# Autodesk Inventor assembly: 1376.000(1)
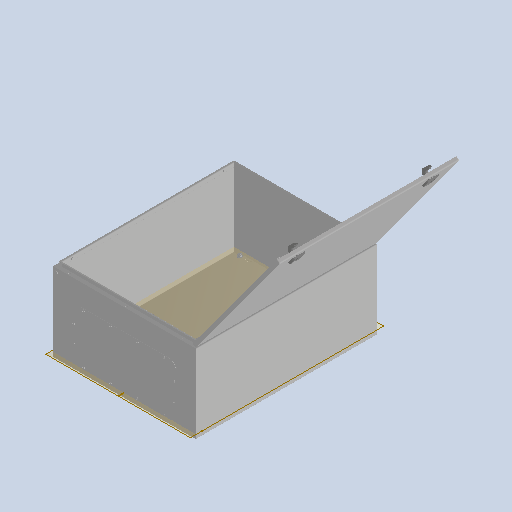
[picture p0: Inventor's stored thumbnail of the model, 512x512]
Saved by Autodesk Inventor 2025.2 (Build 292293000, 293)
## iProperties
Created: 2025-05-05
Part Number: 1376.000(1)
Catalog Web Link: www.cadenas.de
Description: AX Compact enclosure-sheet steel
Vendor: RITTAL
Document SubType Name: Assembly
Designer: psAdmin
Manufacturer: RITTAL
Mass: 34000 g
Surface Area: 49007 cm^2
Volume: 4441.12 cm^3
Density: 7.65572 g/cm^3
Category: PARTsolutions
Company: RITTAL
PSOL_IDENT_0: {$CADENAS_DATA/23d-libs/rittal/schaltschranksys/kompakt_schaltschr/ae_2_0_asmtab.prj},203 {VTYP=3D},
PSOL_IDENT_1: {STYP=ASSTAB},{NB=1376.000(1)},{LINA=1376.000(1)},{NN=AX Compact enclosure},{DATE=28.04.2025 21:11:2
PSOL_IDENT_2: 3},{GEOMDATE=11.04.2025 11:21:44},{VERSION=},{LINEID=320},{WBVAR=DETAIL},{WBNUMERIC=DETAIL}  {NB=137
PSOL_IDENT_3: 6.000(1)},{LINA=1376.000(1)},{KT=DUMMY},{BEST=1376.000},{BEM=2},{DETAIL=1},{INFOWWW=Website},{BEZ1=A
PSOL_IDENT_4: X Kompakt-Schaltschrank},{BEZ2=Stahlblech},{BEZ3=eintürig},{INFO=Überarbeitete Version 11/2024},{B=6
PSOL_IDENT_5: 00},{H=760},{T=350},{F=550},{G=735},{B1=600},{H1=760},{T1=350},{F1=550},{G1=735},{S=3.0},{ST=MIN},{G
PSOL_IDENT_6: EW=34},{VERS=19},{CNSECLASS51=27-18-01-02},{CNSECLASS70=27-18-01-01},{CNSECLASS80=27-18-01-01},{CNSE
PSOL_IDENT_7: TIM40=EC000261},{PPATH=assemblies_ae_2_0/ae_2_0_asmtpl.prj},{INFOPAGE=ax_s30},{INFOPATH=http://www.r
PSOL_IDENT_8: ittal.com/de-de/part/1376000},{BESTE1=1376},{BESTE2=000},{DETAIL1= 2, 'niedrig', 'detail_2.png', 1, '
PSOL_IDENT_9: hoch', 'detail_1.png', 11  , 'hochsperr', 'detail_11.png'},{CNSETIM80=EC000261},{CNSETIM90=EC000261}
PSOL_IDENT_10: ,{CNSECLASS60=27-18-01-01},{UNSPSC=31-26-15-02}
NB: 1376.000(1)
NN: AX Compact enclosure
NT: sheet steel
NBSYN: $BEST.($DETAIL.)
LINA: 1376.000(1)
CATALOG: Rittal
BEST: 1376.000
DETAIL: high
INFOWWW: webseite
BEZ1: AX Compact enclosure
BEZ2: sheet steel
BEZ3: single door
INFO: Revised version 11/2024
B: 600
H: 760
T: 350
F: 550
G: 735
GEW: 34
CNSECLASS70: 27-18-01-01
CNSECLASS80: 27-18-01-01
CNSETIM80: EC000261
CNSETIM90: EC000261
CNSECLASS60: 27-18-01-01
UNSPSC: 31-26-15-02
SUPPLIER: RITTAL
ARTICLENO: 1376.000(1)
BOMINFO: 1376.000(1)
CREATOR: CADENAS GmbH
Title: 1376.000(1)
Author: Cadenas PARTsolutions
Comments: sheet steel
## Documents named in this file (13)
- C:\Users\lucas\OneDrive\Documentos\Documentos\Gustavo\Mozangao\Projeto Base (5140)\Q.E - Braço Robotico\Q.E Rital\AIS2024\1376_000_1_\1376_000(1).iam
- C:\Users\lucas\OneDrive\Documentos\Documentos\Gustavo\Mozangao\Projeto Base (5140)\Q.E - Braço Robotico\Q.E Rital\AIS2024\1376_000_1_\1376_000(1)_P1.ipt
- C:\Users\lucas\OneDrive\Documentos\Documentos\Gustavo\Mozangao\Projeto Base (5140)\Q.E - Braço Robotico\Q.E Rital\AIS2024\1376_000_1_\1XXX_01_04(B,1)_P7.ipt
- C:\Users\lucas\OneDrive\Documentos\Documentos\Gustavo\Mozangao\Projeto Base (5140)\Q.E - Braço Robotico\Q.E Rital\AIS2024\1376_000_1_\1XXX_01_04(T,1)_P7.ipt
- C:\Users\lucas\OneDrive\Documentos\Documentos\Gustavo\Mozangao\Projeto Base (5140)\Q.E - Braço Robotico\Q.E Rital\AIS2024\1376_000_1_\1676X_01_01(1)_P2.ipt
- C:\Users\lucas\OneDrive\Documentos\Documentos\Gustavo\Mozangao\Projeto Base (5140)\Q.E - Braço Robotico\Q.E Rital\AIS2024\1376_000_1_\6321_050_P9 1.ipt
- C:\Users\lucas\OneDrive\Documentos\Documentos\Gustavo\Mozangao\Projeto Base (5140)\Q.E - Braço Robotico\Q.E Rital\AIS2024\1376_000_1_\1XXX_01_05(1)_P8.ipt
- C:\Users\lucas\OneDrive\Documentos\Documentos\Gustavo\Mozangao\Projeto Base (5140)\Q.E - Braço Robotico\Q.E Rital\AIS2024\1376_000_1_\0000-00186369(1).ipt
- C:\Users\lucas\OneDrive\Documentos\Documentos\Gustavo\Mozangao\Projeto Base (5140)\Q.E - Braço Robotico\Q.E Rital\AIS2024\1376_000_1_\1XX1_04_00_1(1)_P5.ipt
- C:\Users\lucas\OneDrive\Documentos\Documentos\Gustavo\Mozangao\Projeto Base (5140)\Q.E - Braço Robotico\Q.E Rital\AIS2024\1376_000_1_\0000-00082819_P2.ipt
- C:\Users\lucas\OneDrive\Documentos\Documentos\Gustavo\Mozangao\Projeto Base (5140)\Q.E - Braço Robotico\Q.E Rital\AIS2024\1376_000_1_\1676X_02_00_P6_(1).ipt
- C:\Users\lucas\OneDrive\Documentos\Documentos\Gustavo\Mozangao\Projeto Base (5140)\Q.E - Braço Robotico\Q.E Rital\AIS2024\1376_000_1_\0000-00168553(1).ipt
- C:\Users\lucas\OneDrive\Documentos\Documentos\Gustavo\Mozangao\Projeto Base (5140)\Q.E - Braço Robotico\Q.E Rital\AIS2024\1376_000_1_\0000-00189079(1).ipt
## Components (28 placed, 12 different names)
1. 1376_000(1)_P1:1 — SCRO_XY@1 <-> SC_XY@2, SCRO_Z@1 <-> SC_Z@2, SCRO_YZ@1 <-> SC_YZ@2, SCRU_XY@1 <-> SC_XY@3, SCRU_Z@1 <-> SC_Z@3, SCRU_YZ@1 <-> SC_YZ@3, SCLO_XY@1 <-> Hinge_Plug_XY@8, SCLO_Z@1 <-> Hinge_Plug_Z@8, SCLO_YZ@1 <-> Hinge_Plug_YZ@8, SCLU_XY@1 <-> Hinge_Plug_XY@9, SCLU_Z@1 <-> Hinge_Plug_Z@9, SCLU_YZ@1 <-> Hinge_Plug_YZ@9, FP1_XY@1 <-> FP_XY@10, FP1_Z@1 <-> FP_Z@10, FP1_YZ@1 <-> FP_YZ@10, MP_XY@1 <-> MP_XY@23, MP_Z@1 <-> MP_Z@23, MP_YZ@1 <-> MP_YZ@23, to_Plug_XY@1 <-> P1_XY@24, to_Plug_Z@1 <-> P1_Z@24, to_Plug_YZ@1 <-> P1_YZ@24, to_Cap_1_XY@1 <-> CAP_XY@25, to_Cap_1_Z@1 <-> CAP_Z@25, to_Cap_1_YZ@1 <-> CAP_YZ@25, to_Cap_2_XY@1 <-> CAP_XY@26, to_Cap_2_Z@1 <-> CAP_Z@26, to_Cap_2_YZ@1 <-> CAP_YZ@26, to_Cap_3_XY@1 <-> CAP_XY@27, to_Cap_3_Z@1 <-> CAP_Z@27, to_Cap_3_YZ@1 <-> CAP_YZ@27, to_Cap_4_XY@1 <-> CAP_XY@28, to_Cap_4_Z@1 <-> CAP_Z@28, to_Cap_4_YZ@1 <-> CAP_YZ@28
2. 1XXX_01_04(B,1)_P7:1 — SCRO_XY@1 <-> SC_XY@2, SCRO_Z@1 <-> SC_Z@2, SCRO_YZ@1 <-> SC_YZ@2
3. 1XXX_01_04(T,1)_P7:1 — SCRU_XY@1 <-> SC_XY@3, SCRU_Z@1 <-> SC_Z@3, SCRU_YZ@1 <-> SC_YZ@3, TUER2_XY@3 <-> ET_XY@4, TUER2_Z@3 <-> ET_Z@4
4. 1676X_01_01(1)_P2:1 — TUER2_XY@3 <-> ET_XY@4, TUER2_Z@3 <-> ET_Z@4, to_Auflaufelement_XY@4 <-> P9_XY@5, to_Auflaufelement_Z@4 <-> P9_Z@5, to_Auflaufelement_YZ@4 <-> P9_YZ@5, VV1_XY@4 <-> VV_XY@6, VV1_Z@4 <-> VV_Z@6, VV1_YZ@4 <-> VV_YZ@6, VV2_XY@4 <-> VV_XY@7, VV2_Z@4 <-> VV_Z@7, VV2_YZ@4 <-> VV_YZ@7
5. 6321_050_P9 1:1 — to_Auflaufelement_XY@4 <-> P9_XY@5, to_Auflaufelement_Z@4 <-> P9_Z@5, to_Auflaufelement_YZ@4 <-> P9_YZ@5
6. 1XXX_01_05(1)_P8:1 — VV1_XY@4 <-> VV_XY@6, VV1_Z@4 <-> VV_Z@6, VV1_YZ@4 <-> VV_YZ@6
7. 1XXX_01_05(1)_P8:2 — VV2_XY@4 <-> VV_XY@7, VV2_Z@4 <-> VV_Z@7, VV2_YZ@4 <-> VV_YZ@7
8. 0000-00186369(1):1 — SCLO_XY@1 <-> Hinge_Plug_XY@8, SCLO_Z@1 <-> Hinge_Plug_Z@8, SCLO_YZ@1 <-> Hinge_Plug_YZ@8
9. 0000-00186369(1):2 — SCLU_XY@1 <-> Hinge_Plug_XY@9, SCLU_Z@1 <-> Hinge_Plug_Z@9, SCLU_YZ@1 <-> Hinge_Plug_YZ@9
10. 1XX1_04_00_1(1)_P5:1 — FP1_XY@1 <-> FP_XY@10, FP1_Z@1 <-> FP_Z@10, FP1_YZ@1 <-> FP_YZ@10, to_Bolt_1_XY@10 <-> Bolt_XY@11, to_Bolt_1_Z@10 <-> Bolt_Z@11, to_Bolt_1_YZ@10 <-> Bolt_YZ@11, to_Bolt_2_XY@10 <-> Bolt_XY@12, to_Bolt_2_Z@10 <-> Bolt_Z@12, to_Bolt_2_YZ@10 <-> Bolt_YZ@12, to_Bolt_3_XY@10 <-> Bolt_XY@13, to_Bolt_3_Z@10 <-> Bolt_Z@13, to_Bolt_3_YZ@10 <-> Bolt_YZ@13, to_Bolt_4_XY@10 <-> Bolt_XY@14, to_Bolt_4_Z@10 <-> Bolt_Z@14, to_Bolt_4_YZ@10 <-> Bolt_YZ@14, to_Bolt_1_1_XY@10 <-> Bolt_XY@15, to_Bolt_1_1_Z@10 <-> Bolt_Z@15, to_Bolt_1_1_YZ@10 <-> Bolt_YZ@15, to_Bolt_1_2_XY@10 <-> Bolt_XY@16, to_Bolt_1_2_Z@10 <-> Bolt_Z@16, to_Bolt_1_2_YZ@10 <-> Bolt_YZ@16, to_Bolt_1_3_XY@10 <-> Bolt_XY@17, to_Bolt_1_3_Z@10 <-> Bolt_Z@17, to_Bolt_1_3_YZ@10 <-> Bolt_YZ@17, to_Bolt_1_4_XY@10 <-> Bolt_XY@18, to_Bolt_1_4_Z@10 <-> Bolt_Z@18, to_Bolt_1_4_YZ@10 <-> Bolt_YZ@18, to_Bolt_1_5_XY@10 <-> Bolt_XY@19, to_Bolt_1_5_Z@10 <-> Bolt_Z@19, to_Bolt_1_5_YZ@10 <-> Bolt_YZ@19, to_Bolt_1_6_XY@10 <-> Bolt_XY@20, to_Bolt_1_6_Z@10 <-> Bolt_Z@20, to_Bolt_1_6_YZ@10 <-> Bolt_YZ@20, to_Bolt_1_7_XY@10 <-> Bolt_XY@21, to_Bolt_1_7_Z@10 <-> Bolt_Z@21, to_Bolt_1_7_YZ@10 <-> Bolt_YZ@21, to_Bolt_1_8_XY@10 <-> Bolt_XY@22, to_Bolt_1_8_Z@10 <-> Bolt_Z@22, to_Bolt_1_8_YZ@10 <-> Bolt_YZ@22
11. 0000-00082819_P2:1 — to_Bolt_1_XY@10 <-> Bolt_XY@11, to_Bolt_1_Z@10 <-> Bolt_Z@11, to_Bolt_1_YZ@10 <-> Bolt_YZ@11
12. 0000-00082819_P2:2 — to_Bolt_2_XY@10 <-> Bolt_XY@12, to_Bolt_2_Z@10 <-> Bolt_Z@12, to_Bolt_2_YZ@10 <-> Bolt_YZ@12
13. 0000-00082819_P2:3 — to_Bolt_3_XY@10 <-> Bolt_XY@13, to_Bolt_3_Z@10 <-> Bolt_Z@13, to_Bolt_3_YZ@10 <-> Bolt_YZ@13
14. 0000-00082819_P2:4 — to_Bolt_4_XY@10 <-> Bolt_XY@14, to_Bolt_4_Z@10 <-> Bolt_Z@14, to_Bolt_4_YZ@10 <-> Bolt_YZ@14
15. 0000-00082819_P2:5 — to_Bolt_1_1_XY@10 <-> Bolt_XY@15, to_Bolt_1_1_Z@10 <-> Bolt_Z@15, to_Bolt_1_1_YZ@10 <-> Bolt_YZ@15
16. 0000-00082819_P2:6 — to_Bolt_1_2_XY@10 <-> Bolt_XY@16, to_Bolt_1_2_Z@10 <-> Bolt_Z@16, to_Bolt_1_2_YZ@10 <-> Bolt_YZ@16
17. 0000-00082819_P2:7 — to_Bolt_1_3_XY@10 <-> Bolt_XY@17, to_Bolt_1_3_Z@10 <-> Bolt_Z@17, to_Bolt_1_3_YZ@10 <-> Bolt_YZ@17
18. 0000-00082819_P2:8 — to_Bolt_1_4_XY@10 <-> Bolt_XY@18, to_Bolt_1_4_Z@10 <-> Bolt_Z@18, to_Bolt_1_4_YZ@10 <-> Bolt_YZ@18
19. 0000-00082819_P2:9 — to_Bolt_1_5_XY@10 <-> Bolt_XY@19, to_Bolt_1_5_Z@10 <-> Bolt_Z@19, to_Bolt_1_5_YZ@10 <-> Bolt_YZ@19
20. 0000-00082819_P2:10 — to_Bolt_1_6_XY@10 <-> Bolt_XY@20, to_Bolt_1_6_Z@10 <-> Bolt_Z@20, to_Bolt_1_6_YZ@10 <-> Bolt_YZ@20
21. 0000-00082819_P2:11 — to_Bolt_1_7_XY@10 <-> Bolt_XY@21, to_Bolt_1_7_Z@10 <-> Bolt_Z@21, to_Bolt_1_7_YZ@10 <-> Bolt_YZ@21
22. 0000-00082819_P2:12 — to_Bolt_1_8_XY@10 <-> Bolt_XY@22, to_Bolt_1_8_Z@10 <-> Bolt_Z@22, to_Bolt_1_8_YZ@10 <-> Bolt_YZ@22
23. 1676X_02_00_P6_(1):1 — MP_XY@1 <-> MP_XY@23, MP_Z@1 <-> MP_Z@23, MP_YZ@1 <-> MP_YZ@23
24. 0000-00168553(1):1 — to_Plug_XY@1 <-> P1_XY@24, to_Plug_Z@1 <-> P1_Z@24, to_Plug_YZ@1 <-> P1_YZ@24
25. 0000-00189079(1):1 — to_Cap_1_XY@1 <-> CAP_XY@25, to_Cap_1_Z@1 <-> CAP_Z@25, to_Cap_1_YZ@1 <-> CAP_YZ@25
26. 0000-00189079(1):2 — to_Cap_2_XY@1 <-> CAP_XY@26, to_Cap_2_Z@1 <-> CAP_Z@26, to_Cap_2_YZ@1 <-> CAP_YZ@26
27. 0000-00189079(1):3 — to_Cap_3_XY@1 <-> CAP_XY@27, to_Cap_3_Z@1 <-> CAP_Z@27, to_Cap_3_YZ@1 <-> CAP_YZ@27
28. 0000-00189079(1):4 — to_Cap_4_XY@1 <-> CAP_XY@28, to_Cap_4_Z@1 <-> CAP_Z@28, to_Cap_4_YZ@1 <-> CAP_YZ@28
## Relationships (80: Mate 53, Angle 26, Flush 1)
- SCRO_XY@1 <-> SC_XY@2 [Mate]: 1376_000(1)_P1:1 ↔ 1XXX_01_04(B,1)_P7:1
- SCRO_Z@1 <-> SC_Z@2 [Mate]: 1376_000(1)_P1:1 ↔ 1XXX_01_04(B,1)_P7:1
- SCRO_YZ@1 <-> SC_YZ@2 [Angle] (0 deg): 1376_000(1)_P1:1 ↔ 1XXX_01_04(B,1)_P7:1
- SCRU_XY@1 <-> SC_XY@3 [Mate]: 1376_000(1)_P1:1 ↔ 1XXX_01_04(T,1)_P7:1
- SCRU_Z@1 <-> SC_Z@3 [Mate]: 1376_000(1)_P1:1 ↔ 1XXX_01_04(T,1)_P7:1
- SCRU_YZ@1 <-> SC_YZ@3 [Angle] (0 deg): 1376_000(1)_P1:1 ↔ 1XXX_01_04(T,1)_P7:1
- TUER2_XY@3 <-> ET_XY@4 [Mate]: 1XXX_01_04(T,1)_P7:1 ↔ 1676X_01_01(1)_P2:1
- TUER2_Z@3 <-> ET_Z@4 [Mate]: 1XXX_01_04(T,1)_P7:1 ↔ 1676X_01_01(1)_P2:1
- to_Auflaufelement_XY@4 <-> P9_XY@5 [Mate]: 1676X_01_01(1)_P2:1 ↔ 6321_050_P9 1:1
- to_Auflaufelement_Z@4 <-> P9_Z@5 [Mate]: 1676X_01_01(1)_P2:1 ↔ 6321_050_P9 1:1
- to_Auflaufelement_YZ@4 <-> P9_YZ@5 [Angle] (180 deg): 1676X_01_01(1)_P2:1 ↔ 6321_050_P9 1:1
- VV1_XY@4 <-> VV_XY@6 [Mate]: 1676X_01_01(1)_P2:1 ↔ 1XXX_01_05(1)_P8:1
- VV1_Z@4 <-> VV_Z@6 [Mate]: 1676X_01_01(1)_P2:1 ↔ 1XXX_01_05(1)_P8:1
- VV1_YZ@4 <-> VV_YZ@6 [Angle] (0 deg): 1676X_01_01(1)_P2:1 ↔ 1XXX_01_05(1)_P8:1
- VV2_XY@4 <-> VV_XY@7 [Mate]: 1676X_01_01(1)_P2:1 ↔ 1XXX_01_05(1)_P8:2
- VV2_Z@4 <-> VV_Z@7 [Mate]: 1676X_01_01(1)_P2:1 ↔ 1XXX_01_05(1)_P8:2
- VV2_YZ@4 <-> VV_YZ@7 [Angle] (0 deg): 1676X_01_01(1)_P2:1 ↔ 1XXX_01_05(1)_P8:2
- SCLO_XY@1 <-> Hinge_Plug_XY@8 [Mate] (1.5 mm): 1376_000(1)_P1:1 ↔ 0000-00186369(1):1
- SCLO_Z@1 <-> Hinge_Plug_Z@8 [Mate]: 1376_000(1)_P1:1 ↔ 0000-00186369(1):1
- SCLO_YZ@1 <-> Hinge_Plug_YZ@8 [Angle] (0 deg): 1376_000(1)_P1:1 ↔ 0000-00186369(1):1
- SCLU_XY@1 <-> Hinge_Plug_XY@9 [Mate] (1.5 mm): 1376_000(1)_P1:1 ↔ 0000-00186369(1):2
- SCLU_Z@1 <-> Hinge_Plug_Z@9 [Mate]: 1376_000(1)_P1:1 ↔ 0000-00186369(1):2
- SCLU_YZ@1 <-> Hinge_Plug_YZ@9 [Angle] (0 deg): 1376_000(1)_P1:1 ↔ 0000-00186369(1):2
- FP1_XY@1 <-> FP_XY@10 [Mate]: 1376_000(1)_P1:1 ↔ 1XX1_04_00_1(1)_P5:1
- FP1_Z@1 <-> FP_Z@10 [Mate]: 1376_000(1)_P1:1 ↔ 1XX1_04_00_1(1)_P5:1
- FP1_YZ@1 <-> FP_YZ@10 [Angle] (0 deg): 1376_000(1)_P1:1 ↔ 1XX1_04_00_1(1)_P5:1
- to_Bolt_1_XY@10 <-> Bolt_XY@11 [Mate]: 1XX1_04_00_1(1)_P5:1 ↔ 0000-00082819_P2:1
- to_Bolt_1_Z@10 <-> Bolt_Z@11 [Mate]: 1XX1_04_00_1(1)_P5:1 ↔ 0000-00082819_P2:1
- to_Bolt_1_YZ@10 <-> Bolt_YZ@11 [Angle] (0 deg): 1XX1_04_00_1(1)_P5:1 ↔ 0000-00082819_P2:1
- to_Bolt_2_XY@10 <-> Bolt_XY@12 [Mate]: 1XX1_04_00_1(1)_P5:1 ↔ 0000-00082819_P2:2
- to_Bolt_2_Z@10 <-> Bolt_Z@12 [Mate]: 1XX1_04_00_1(1)_P5:1 ↔ 0000-00082819_P2:2
- to_Bolt_2_YZ@10 <-> Bolt_YZ@12 [Angle] (0 deg): 1XX1_04_00_1(1)_P5:1 ↔ 0000-00082819_P2:2
- to_Bolt_3_XY@10 <-> Bolt_XY@13 [Mate]: 1XX1_04_00_1(1)_P5:1 ↔ 0000-00082819_P2:3
- to_Bolt_3_Z@10 <-> Bolt_Z@13 [Mate]: 1XX1_04_00_1(1)_P5:1 ↔ 0000-00082819_P2:3
- to_Bolt_3_YZ@10 <-> Bolt_YZ@13 [Angle] (0 deg): 1XX1_04_00_1(1)_P5:1 ↔ 0000-00082819_P2:3
- to_Bolt_4_XY@10 <-> Bolt_XY@14 [Mate]: 1XX1_04_00_1(1)_P5:1 ↔ 0000-00082819_P2:4
- to_Bolt_4_Z@10 <-> Bolt_Z@14 [Mate]: 1XX1_04_00_1(1)_P5:1 ↔ 0000-00082819_P2:4
- to_Bolt_4_YZ@10 <-> Bolt_YZ@14 [Angle] (0 deg): 1XX1_04_00_1(1)_P5:1 ↔ 0000-00082819_P2:4
- to_Bolt_1_1_XY@10 <-> Bolt_XY@15 [Mate]: 1XX1_04_00_1(1)_P5:1 ↔ 0000-00082819_P2:5
- to_Bolt_1_1_Z@10 <-> Bolt_Z@15 [Mate]: 1XX1_04_00_1(1)_P5:1 ↔ 0000-00082819_P2:5
- to_Bolt_1_1_YZ@10 <-> Bolt_YZ@15 [Angle] (0 deg): 1XX1_04_00_1(1)_P5:1 ↔ 0000-00082819_P2:5
- to_Bolt_1_2_XY@10 <-> Bolt_XY@16 [Mate]: 1XX1_04_00_1(1)_P5:1 ↔ 0000-00082819_P2:6
- to_Bolt_1_2_Z@10 <-> Bolt_Z@16 [Mate]: 1XX1_04_00_1(1)_P5:1 ↔ 0000-00082819_P2:6
- to_Bolt_1_2_YZ@10 <-> Bolt_YZ@16 [Angle] (0 deg): 1XX1_04_00_1(1)_P5:1 ↔ 0000-00082819_P2:6
- to_Bolt_1_3_XY@10 <-> Bolt_XY@17 [Mate]: 1XX1_04_00_1(1)_P5:1 ↔ 0000-00082819_P2:7
- to_Bolt_1_3_Z@10 <-> Bolt_Z@17 [Mate]: 1XX1_04_00_1(1)_P5:1 ↔ 0000-00082819_P2:7
- to_Bolt_1_3_YZ@10 <-> Bolt_YZ@17 [Angle] (0 deg): 1XX1_04_00_1(1)_P5:1 ↔ 0000-00082819_P2:7
- to_Bolt_1_4_XY@10 <-> Bolt_XY@18 [Mate]: 1XX1_04_00_1(1)_P5:1 ↔ 0000-00082819_P2:8
- to_Bolt_1_4_Z@10 <-> Bolt_Z@18 [Mate]: 1XX1_04_00_1(1)_P5:1 ↔ 0000-00082819_P2:8
- to_Bolt_1_4_YZ@10 <-> Bolt_YZ@18 [Angle] (0 deg): 1XX1_04_00_1(1)_P5:1 ↔ 0000-00082819_P2:8
- to_Bolt_1_5_XY@10 <-> Bolt_XY@19 [Mate]: 1XX1_04_00_1(1)_P5:1 ↔ 0000-00082819_P2:9
- to_Bolt_1_5_Z@10 <-> Bolt_Z@19 [Mate]: 1XX1_04_00_1(1)_P5:1 ↔ 0000-00082819_P2:9
- to_Bolt_1_5_YZ@10 <-> Bolt_YZ@19 [Angle] (0 deg): 1XX1_04_00_1(1)_P5:1 ↔ 0000-00082819_P2:9
- to_Bolt_1_6_XY@10 <-> Bolt_XY@20 [Mate]: 1XX1_04_00_1(1)_P5:1 ↔ 0000-00082819_P2:10
- to_Bolt_1_6_Z@10 <-> Bolt_Z@20 [Mate]: 1XX1_04_00_1(1)_P5:1 ↔ 0000-00082819_P2:10
- to_Bolt_1_6_YZ@10 <-> Bolt_YZ@20 [Angle] (0 deg): 1XX1_04_00_1(1)_P5:1 ↔ 0000-00082819_P2:10
- to_Bolt_1_7_XY@10 <-> Bolt_XY@21 [Mate]: 1XX1_04_00_1(1)_P5:1 ↔ 0000-00082819_P2:11
- to_Bolt_1_7_Z@10 <-> Bolt_Z@21 [Mate]: 1XX1_04_00_1(1)_P5:1 ↔ 0000-00082819_P2:11
- to_Bolt_1_7_YZ@10 <-> Bolt_YZ@21 [Angle] (0 deg): 1XX1_04_00_1(1)_P5:1 ↔ 0000-00082819_P2:11
- to_Bolt_1_8_XY@10 <-> Bolt_XY@22 [Mate]: 1XX1_04_00_1(1)_P5:1 ↔ 0000-00082819_P2:12
- to_Bolt_1_8_Z@10 <-> Bolt_Z@22 [Mate]: 1XX1_04_00_1(1)_P5:1 ↔ 0000-00082819_P2:12
- to_Bolt_1_8_YZ@10 <-> Bolt_YZ@22 [Angle] (0 deg): 1XX1_04_00_1(1)_P5:1 ↔ 0000-00082819_P2:12
- MP_XY@1 <-> MP_XY@23 [Mate]: 1376_000(1)_P1:1 ↔ 1676X_02_00_P6_(1):1
- MP_Z@1 <-> MP_Z@23 [Mate]: 1376_000(1)_P1:1 ↔ 1676X_02_00_P6_(1):1
- MP_YZ@1 <-> MP_YZ@23 [Angle] (0 deg): 1376_000(1)_P1:1 ↔ 1676X_02_00_P6_(1):1
- to_Plug_XY@1 <-> P1_XY@24 [Flush]: 1376_000(1)_P1:1 ↔ 0000-00168553(1):1
- to_Plug_Z@1 <-> P1_Z@24 [Mate]: 1376_000(1)_P1:1 ↔ 0000-00168553(1):1
- to_Plug_YZ@1 <-> P1_YZ@24 [Angle] (0 deg): 1376_000(1)_P1:1 ↔ 0000-00168553(1):1
- to_Cap_1_XY@1 <-> CAP_XY@25 [Mate] (-1.55 mm): 1376_000(1)_P1:1 ↔ 0000-00189079(1):1
- to_Cap_1_Z@1 <-> CAP_Z@25 [Mate]: 1376_000(1)_P1:1 ↔ 0000-00189079(1):1
- to_Cap_1_YZ@1 <-> CAP_YZ@25 [Angle] (0 deg): 1376_000(1)_P1:1 ↔ 0000-00189079(1):1
- to_Cap_2_XY@1 <-> CAP_XY@26 [Mate] (-1.55 mm): 1376_000(1)_P1:1 ↔ 0000-00189079(1):2
- to_Cap_2_Z@1 <-> CAP_Z@26 [Mate]: 1376_000(1)_P1:1 ↔ 0000-00189079(1):2
- to_Cap_2_YZ@1 <-> CAP_YZ@26 [Angle] (0 deg): 1376_000(1)_P1:1 ↔ 0000-00189079(1):2
- to_Cap_3_XY@1 <-> CAP_XY@27 [Mate] (-1.55 mm): 1376_000(1)_P1:1 ↔ 0000-00189079(1):3
- to_Cap_3_Z@1 <-> CAP_Z@27 [Mate]: 1376_000(1)_P1:1 ↔ 0000-00189079(1):3
- to_Cap_3_YZ@1 <-> CAP_YZ@27 [Angle] (0 deg): 1376_000(1)_P1:1 ↔ 0000-00189079(1):3
- to_Cap_4_XY@1 <-> CAP_XY@28 [Mate] (-1.55 mm): 1376_000(1)_P1:1 ↔ 0000-00189079(1):4
- to_Cap_4_Z@1 <-> CAP_Z@28 [Mate]: 1376_000(1)_P1:1 ↔ 0000-00189079(1):4
- to_Cap_4_YZ@1 <-> CAP_YZ@28 [Angle] (0 deg): 1376_000(1)_P1:1 ↔ 0000-00189079(1):4
